# Autodesk Inventor assembly: дрон сборка
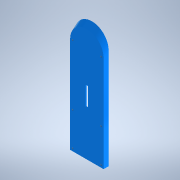
[picture p0: Inventor's stored thumbnail of the model, 180x180]
Saved by Autodesk Inventor 2022.1 (Build 261234000, 234)
## iProperties
Created: 2021-12-25
Part Number: дрон сборка
Document SubType Name: Assembly
Designer: Grigori
Author: Grigori
## Documents named in this file (14)
- C:\Users\Grigo\Desktop\Дрон\Сборка\сборка низ.iam
- C:\Users\Grigo\Desktop\Дрон\Сборка\корпус.ipt
- C:\Users\Grigo\Desktop\Дрон\Сборка\APM 2.5 Side Entry Case.ipt
- C:\Users\Grigo\Desktop\Дрон\Сборка\PX4 Neo M8N GPS.ipt
- C:\Users\Grigo\Desktop\Дрон\Сборка\3D Robotics Radio Telemetry Kit.ipt
- C:\Users\User\Documents\GitHub\ModularDrone\PartsModels\Box Battery\Сборка.ipt
- C:\Users\Grigo\Desktop\Дрон\Сборка\Крышка на отсек с батареей.ipt
- C:\Users\Grigo\Documents\Inventor\Content Center Files\R2022\ru-RU\AS 1427(01)\AS 1427 - M3 x 10(3).ipt
- C:\Users\Grigo\Desktop\Дрон\Сборка\Сборка крышка.iam
- C:\Users\User\Documents\Inventor\Content Center Files\R2022\ru-RU\DIN 976-1 A\DIN 976-1 - M5 x 60 - A.ipt
- C:\Users\Grigo\Desktop\Дрон\Сборка\площадка.ipt
- C:\Users\Grigo\Desktop\Дрон\Сборка\проставка.ipt
- C:\Users\Grigo\Desktop\Дрон\Сборка\power boars scheme v3.iam
- C:\Users\User\Documents\Inventor\Content Center Files\R2022\ru-RU\ANSI B 18.2.4.1 M(1)\ANSI B 18.2.4.1 M - M4 x 0,7Style 1.ipt
## Components (35 placed, 13 different names)
1. корпус:1 — Совмещение:1, Совмещение:2, Совмещение:3, С поворотом:1, С поворотом:2, Совмещение:4, Совмещение:5, Совмещение:6, Вставка:1, Вставка:2, Вставка:3, Вставка:4, Вставка:5
2. APM 2.5 Side Entry Case:1 — Жесткий:7
3. PX4 Neo M8N GPS:1 — Жесткий:9
4. 3D Robotics Radio Telemetry Kit:1 — Жесткий:8
5. Сборка:1 — Совмещение:1, Совмещение:2, Совмещение:3
6. Крышка на отсек с батареей:1 — С поворотом:1, С поворотом:2, С поворотом:3, С поворотом:4, Жесткий:2, С поворотом:5, Жесткий:3, Жесткий:4, Жесткий:5, Жесткий:6
7. AS 1427 - метрическая M3 x 10:1 — Жесткий:3
8. AS 1427 - метрическая M3 x 10:2 — Жесткий:2
9. AS 1427 - метрическая M3 x 10:3 — С поворотом:4
10. AS 1427 - метрическая M3 x 10:4 — Жесткий:5
11. AS 1427 - метрическая M3 x 10:5 — Жесткий:6
12. AS 1427 - метрическая M3 x 10:6 — С поворотом:5
13. AS 1427 - метрическая M3 x 10:7 — Жесткий:4
14. AS 1427 - метрическая M3 x 10:8 — С поворотом:3
15. Сборка крышка:1 [sub-assembly] — Совмещение:4, Совмещение:5, Совмещение:6
16. DIN 976-1 A M5 x 60:1 — Вставка:1, Вставка:7, Вставка:13
17. DIN 976-1 A M5 x 60:2 — Вставка:2, Вставка:6, Вставка:14
18. DIN 976-1 A M5 x 60:3 — Вставка:3, Вставка:8, Вставка:12
19. DIN 976-1 A M5 x 60:4 — Вставка:4, Вставка:9, Вставка:11
20. площадка:1 — Вставка:5, Жесткий:7
21. проставка:1 — Вставка:9
22. проставка:2 — Вставка:8
23. проставка:3 — Вставка:7, Вставка:10
24. проставка:4 — Вставка:6
25. площадка:2 — Вставка:10, Жесткий:8, Жесткий:9
26. проставка:5 — Вставка:12
27. проставка:6 — Вставка:13, Вставка:15
28. проставка:7 — Вставка:14
29. проставка:8 — Вставка:11
30. площадка:3 — Вставка:15, Жесткий:10, Вставка:16, Вставка:17, Вставка:18, Вставка:19
31. power boars scheme v3:1 [sub-assembly] — Жесткий:10
32. Шестигранная гайка метрическая M4 x 0,7:1 — Вставка:16
33. Шестигранная гайка метрическая M4 x 0,7:2 — Вставка:17
34. Шестигранная гайка метрическая M4 x 0,7:3 — Вставка:18
35. Шестигранная гайка метрическая M4 x 0,7:4 — Вставка:19
## Relationships (39: Insert 19, WeldJoint 9, Mate 6, RevoluteJoint 5)
- Совмещение:1 [Mate]: корпус:1 ↔ Сборка:1
- Совмещение:2 [Mate]: корпус:1 ↔ Сборка:1
- Совмещение:3 [Mate]: корпус:1 ↔ Сборка:1
- С поворотом:1 [RevoluteJoint]: корпус:1 ↔ Крышка на отсек с батареей:1
- С поворотом:2 [RevoluteJoint]: корпус:1 ↔ Крышка на отсек с батареей:1
- С поворотом:3 [RevoluteJoint]: Крышка на отсек с батареей:1 ↔ AS 1427 - метрическая M3 x 10:8
- С поворотом:4 [RevoluteJoint]: Крышка на отсек с батареей:1 ↔ AS 1427 - метрическая M3 x 10:3
- Жесткий:2 [WeldJoint]: Крышка на отсек с батареей:1 ↔ AS 1427 - метрическая M3 x 10:2
- С поворотом:5 [RevoluteJoint]: Крышка на отсек с батареей:1 ↔ AS 1427 - метрическая M3 x 10:6
- Жесткий:3 [WeldJoint]: Крышка на отсек с батареей:1 ↔ AS 1427 - метрическая M3 x 10:1
- Жесткий:4 [WeldJoint]: Крышка на отсек с батареей:1 ↔ AS 1427 - метрическая M3 x 10:7
- Жесткий:5 [WeldJoint]: Крышка на отсек с батареей:1 ↔ AS 1427 - метрическая M3 x 10:4
- Жесткий:6 [WeldJoint]: Крышка на отсек с батареей:1 ↔ AS 1427 - метрическая M3 x 10:5
- Совмещение:4 [Mate]: корпус:1 ↔ Сборка крышка:1
- Совмещение:5 [Mate]: корпус:1 ↔ Сборка крышка:1
- Совмещение:6 [Mate]: корпус:1 ↔ Сборка крышка:1
- Вставка:1 [Insert] (-46 mm): корпус:1 ↔ DIN 976-1 A M5 x 60:1
- Вставка:2 [Insert] (-46 mm): корпус:1 ↔ DIN 976-1 A M5 x 60:2
- Вставка:3 [Insert] (-46 mm): корпус:1 ↔ DIN 976-1 A M5 x 60:3
- Вставка:4 [Insert] (-46 mm): корпус:1 ↔ DIN 976-1 A M5 x 60:4
- Вставка:5 [Insert]: корпус:1 ↔ площадка:1
- Жесткий:7 [WeldJoint]: APM 2.5 Side Entry Case:1 ↔ площадка:1
- Вставка:6 [Insert] (15 mm): DIN 976-1 A M5 x 60:2 ↔ проставка:4
- Вставка:7 [Insert] (15 mm): DIN 976-1 A M5 x 60:1 ↔ проставка:3
- Вставка:8 [Insert] (15 mm): DIN 976-1 A M5 x 60:3 ↔ проставка:2
- Вставка:9 [Insert] (15 mm): DIN 976-1 A M5 x 60:4 ↔ проставка:1
- Вставка:10 [Insert]: проставка:3 ↔ площадка:2
- Жесткий:8 [WeldJoint]: 3D Robotics Radio Telemetry Kit:1 ↔ площадка:2
- Жесткий:9 [WeldJoint]: PX4 Neo M8N GPS:1 ↔ площадка:2
- Вставка:11 [Insert] (4 mm): DIN 976-1 A M5 x 60:4 ↔ проставка:8
- Вставка:12 [Insert] (4 mm): DIN 976-1 A M5 x 60:3 ↔ проставка:5
- Вставка:13 [Insert] (4 mm): DIN 976-1 A M5 x 60:1 ↔ проставка:6
- Вставка:14 [Insert] (4 mm): DIN 976-1 A M5 x 60:2 ↔ проставка:7
- Вставка:15 [Insert]: проставка:6 ↔ площадка:3
- Жесткий:10 [WeldJoint]: площадка:3 ↔ power boars scheme v3:1
- Вставка:16 [Insert]: площадка:3 ↔ Шестигранная гайка метрическая M4 x 0,7:1
- Вставка:17 [Insert]: площадка:3 ↔ Шестигранная гайка метрическая M4 x 0,7:2
- Вставка:18 [Insert]: площадка:3 ↔ Шестигранная гайка метрическая M4 x 0,7:3
- Вставка:19 [Insert]: площадка:3 ↔ Шестигранная гайка метрическая M4 x 0,7:4
